# Autodesk Inventor assembly: CC1x1
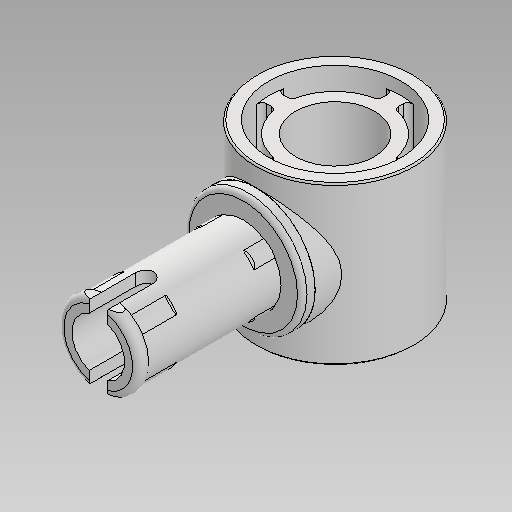
[picture p0: Inventor's stored thumbnail of the model, 512x512]
Saved by Autodesk Inventor 2020 (Build 240168000, 168)
## iProperties
Created: 2019-05-05
Part Number: CC1x1
Document SubType Name: Assembly
Designer: Varga Daniel
Author: Varga Daniel
## Documents named in this file (4)
- C:\!_Dani\!_cloud\OneDrive\!_munka\Revolution\StructuralParts\Connector Boxes\Connector Cubes\CC1x1.iam
- C:\!_Dani\!_cloud\OneDrive\!_munka\Revolution\StructuralParts\Beams\beam_single_1x1_part.ipt
- C:\!_Dani\!_cloud\OneDrive\!_munka\Revolution\StructuralParts\Connector pins\CP1_base\CP1_base-both_sides_anti_skid.ipt
- C:\!_Dani\!_cloud\OneDrive\!_munka\Revolution\StructuralParts\Connector pins\CP1_base.ipt
## Components (2 placed, 2 different names)
1. beam_single_1x1_part:1 — Mate:3, Flush:3, Flush:4
2. CP1_base-both_sides_anti_skid:4 — Mate:3, Flush:3, Flush:4
## Relationships (3: Flush 2, Mate 1)
- Mate:3: beam_single_1x1_part:1 ↔ CP1_base-both_sides_anti_skid:4
- Flush:3: beam_single_1x1_part:1 ↔ CP1_base-both_sides_anti_skid:4
- Flush:4: beam_single_1x1_part:1 ↔ CP1_base-both_sides_anti_skid:4
